# Autodesk Inventor assembly: 70069764
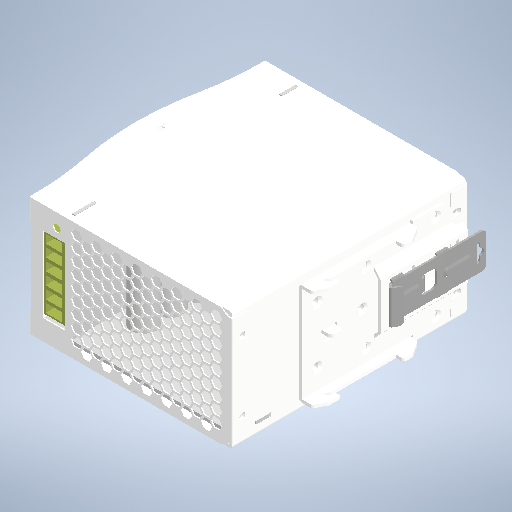
[picture p0: Inventor's stored thumbnail of the model, 512x512]
Saved by Autodesk Inventor 2025.3 (Build 293356000, 356)
## iProperties
Company: TraceParts S.A.
Created: 2026-07-31
Part Number: 70069764
Checked By: TraceParts S.A.
Catalog Web Link: www.traceparts.com
Document SubType Name: Assembly
Designer: TraceParts
Sending System: TraceParts v2
Major Version: 6.0
Minor Version: 0.0
Format Version: 0.0
Product Id: TraceParts v2
REFERENCE: WDR-240-24
SUPPLIER_PART_NUMBER: 70069764
rs_stock_number: 70069764
SUPPLIER_NAME: RS Americas
SUPPLIER: MEAN WELL
DESIGN: WDR-240-24 - Power Supply, AC-DC 24V 10A 240W PFC DIN Rail Mount WDR-240 Series
TraceParts.PartNumber: 90-26072023-080797
TraceParts.PartTitle: WDR-240-24 - Power Supply, AC-DC 24V 10A 240W PFC DIN Rail Mount WDR-240 Series
TraceParts.InstanceId: 90-26072023-08079736FDR7KA1GQNQOJK3QTZMLD2H
TRACEPARTS: TRACEPARTS
TraceParts.PartLanguage: en
TraceParts.PartVersion: 1.0.1
Author: TraceParts
## Documents named in this file (7)
- C:\Users\louis\OneDrive\Desktop\R_Trident\02_CAD\01_Standard_Parts\04_ELE_Electrical_Automation\wdr_240_24\WDR-240-24.iam
- C:\Users\louis\OneDrive\Desktop\R_Trident\02_CAD\01_Standard_Parts\04_ELE_Electrical_Automation\wdr_240_24\70069764_01.ipt
- C:\Users\louis\OneDrive\Desktop\R_Trident\02_CAD\01_Standard_Parts\04_ELE_Electrical_Automation\wdr_240_24\70069764_02.ipt
- C:\Users\louis\OneDrive\Desktop\R_Trident\02_CAD\01_Standard_Parts\04_ELE_Electrical_Automation\wdr_240_24\70069764_03.ipt
- C:\Users\louis\OneDrive\Desktop\R_Trident\02_CAD\01_Standard_Parts\04_ELE_Electrical_Automation\wdr_240_24\70069764_04.ipt
- C:\Users\louis\OneDrive\Desktop\R_Trident\02_CAD\01_Standard_Parts\04_ELE_Electrical_Automation\wdr_240_24\70069764_05.ipt
- C:\Users\louis\OneDrive\Desktop\R_Trident\02_CAD\01_Standard_Parts\04_ELE_Electrical_Automation\wdr_240_24\70069764_06.ipt
## Components (6 placed, 6 different names)
1. 70069764_Temp_1:1
2. 70069764_Temp_2:1 — Flush:1
3. 70069764_Temp_3:1
4. 70069764_Temp_4:1
5. 70069764_Temp_5:1
6. 70069764_Temp_6:1
## Relationships (1: Flush 1)
- Flush:1 (17.5 mm): 70069764_Temp_2:1
